# Autodesk Inventor assembly: MotionBaseGeneric
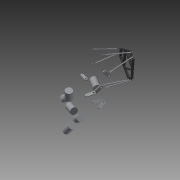
[picture p0: Inventor's stored thumbnail of the model, 180x180]
Saved by Autodesk Inventor 2015 SP1 (Build 190203100, 203)
## iProperties
Created: 2016-02-02
Part Number: MotionBaseGeneric
Document SubType Name: Assembly
Designer: tuttlem
Author: tuttlem
## Documents named in this file (7)
- C:\Users\jonesdm\Desktop\MotionBase\CAD\MotionBaseCAD\MotionBaseGeneric.iam
- C:\Users\jonesdm\Desktop\MotionBase\CAD\MotionBaseCAD\Platform.ipt
- C:\Users\jonesdm\Desktop\MotionBase\CAD\MotionBaseCAD\BasePlatform.ipt
- C:\Users\jonesdm\Desktop\MotionBase\CAD\MotionBaseCAD\Rod.ipt
- C:\Users\jonesdm\Desktop\MotionBase\CAD\MotionBaseCAD\Rod_MIR.ipt
- C:\Users\jonesdm\Desktop\MotionBase\CAD\MotionBaseCAD\arm.ipt
- C:\Users\jonesdm\Desktop\MotionBase\CAD\MotionBaseCAD\Motor.ipt
## Components (26 placed, 6 different names)
1. Platform:1 — Insert:3, Insert:5, Mate:1, Flush:7, Mate:2, Flush:8, Mate:3, Mate:4, Mate:5, Flush:9
2. BasePlatform:1
3. Motor:11
4. Motor:10
5. Motor:9
6. Motor:8
7. Motor:7
8. Motor:1
9. Rod_MIR:1 — Flush:1, Tangent:1
10. Rod_MIR:2
11. Rod_MIR:3
12. Rod_MIR:4
13. Rod_MIR:5
14. Rod_MIR:6
15. Rod:1 — Flush:1, Tangent:1, Insert:3
16. Rod:2 — Insert:5
17. Rod:3 — Mate:1, Flush:7
18. Rod:4 — Mate:2, Flush:8
19. Rod:5 — Mate:3, Mate:4
20. Rod:6 — Mate:5, Flush:9
21. arm:1
22. arm:8
23. arm:9
24. arm:10
25. arm:11
26. arm:12
## Relationships (22: Flush 9, Tangent 6, Mate 5, Insert 2)
- Flush:1: Rod_MIR:1 ↔ Rod:1
- Tangent:1: Rod_MIR:1 ↔ Rod:1
- [Flush]: Rod_MIR:2 ↔ Rod:2
- [Tangent]: Rod_MIR:2 ↔ Rod:2
- Insert:3: Platform:1 ↔ Rod:1
- Insert:5: Platform:1 ↔ Rod:2
- [Flush]: Rod_MIR:3 ↔ Rod:3
- [Tangent]: Rod_MIR:3 ↔ Rod:3
- [Flush]: Rod_MIR:4 ↔ Rod:4
- [Tangent]: Rod_MIR:4 ↔ Rod:4
- [Flush]: Rod_MIR:5 ↔ Rod:5
- [Tangent]: Rod_MIR:5 ↔ Rod:5
- [Flush]: Rod_MIR:6 ↔ Rod:6
- [Tangent]: Rod_MIR:6 ↔ Rod:6
- Mate:1: Platform:1 ↔ Rod:3
- Flush:7: Platform:1 ↔ Rod:3
- Mate:2: Platform:1 ↔ Rod:4
- Flush:8: Platform:1 ↔ Rod:4
- Mate:3: Platform:1 ↔ Rod:5
- Mate:4: Platform:1 ↔ Rod:5
- Mate:5: Platform:1 ↔ Rod:6
- Flush:9: Platform:1 ↔ Rod:6
## Named parameters: d2_d1 = 0 mm, d3_d0 = 0 mm, d18_d1 = 0 mm, d21_d0 = 0 mm, d22_d1 = 0 mm, d25_d0 = 0 mm, d26_d1 = 0 mm, d29_d0 = 0 mm, d30_d1 = 0 mm, d33_d0 = 0 mm
